# Autodesk Inventor assembly: stator
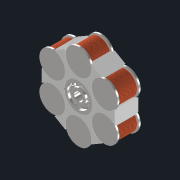
[picture p0: Inventor's stored thumbnail of the model, 180x180]
Saved by Autodesk Inventor 2022.2 (Build 262287010, 287A)
## iProperties
Created: 2023-07-19
Part Number: stator
Document SubType Name: Assembly
Designer: StijnC
Author: StijnC
## Documents named in this file (5)
- C:\Users\techn\Desktop\AFM\V2\stator.iam
- C:\Users\techn\Desktop\AFM\V2\motor15.ipt
- C:\Users\techn\Desktop\AFM\V2\core.ipt
- C:\Users\techn\Desktop\AFM\V2\coil.ipt
- C:\Users\techn\Documents\Inventor\Content Center Files\R2022\en-US\DIN 625 - T1\DIN 625 T1 - 626 - 6 x 19 x 6.ipt
## Components (22 placed, 4 different names)
1. motor15:1 — Mate:1, Mate:2, Mate:3, Mate:6, Mate:7, Flush:1, Mate:30, Flush:2
2. motor15:2 — Mate:2, Mate:3, Mate:4, Mate:5, Angle:1, Flush:1, Mate:29, Flush:3
3. DIN 625 - T1 626 - 6 x 19 x 6:1 — Mate:29, Flush:3
4. DIN 625 - T1 626 - 6 x 19 x 6:2 — Mate:30, Flush:2
5. core:2 — Mate:6, Mate:7
6. core:1 — Mate:4, Mate:5, Mate:28, Tangent:1
7. core:3
8. core:4
9. core:5
10. core:6
11. core:7
12. core:8
13. core:9
14. core:10
15. core:11
16. core:12
17. coil:1 — Mate:28, Tangent:1
18. coil:2
19. coil:3
20. coil:4
21. coil:5
22. coil:6
## Component patterns: (6 elements, first: core:2 + core:1), (6 elements, first: coil:1)
## Relationships (15: Mate 10, Flush 3, Angle 1, Tangent 1)
- Mate:1: motor15:1
- Mate:2: motor15:1 ↔ motor15:2
- Mate:3: motor15:1 ↔ motor15:2
- Mate:4: motor15:2 ↔ core:1
- Mate:5: motor15:2 ↔ core:1
- Mate:6: motor15:1 ↔ core:2
- Mate:7: motor15:1 ↔ core:2
- Angle:1 (0 deg): motor15:2
- Flush:1: motor15:1 ↔ motor15:2
- Mate:28: core:1 ↔ coil:1
- Tangent:1: core:1 ↔ coil:1
- Mate:29: motor15:2 ↔ DIN 625 - T1 626 - 6 x 19 x 6:1
- Mate:30: motor15:1 ↔ DIN 625 - T1 626 - 6 x 19 x 6:2
- Flush:2: motor15:1 ↔ DIN 625 - T1 626 - 6 x 19 x 6:2
- Flush:3: motor15:2 ↔ DIN 625 - T1 626 - 6 x 19 x 6:1
